# Autodesk Inventor assembly: p80 mount assembl
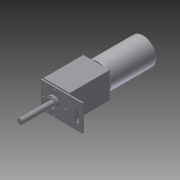
[picture p0: Inventor's stored thumbnail of the model, 180x180]
Saved by Autodesk Inventor 2013 (Build 170138000, 138)
## iProperties
Created: 2013-02-03
Part Number: p80 mount assembl
Document SubType Name: Assembly
Designer: Arpan
Mass: 804.871 g
Surface Area: 938.695 cm^2
Volume: 776.478 cm^3
Density: 1.03657 g/cm^3
Author: Arpan
## Documents named in this file (4)
- C:\Users\Moses\Documents\GitHub\frc2013CAD\Cimber actual\p80 mount assembl.iam
- C:\Users\Moses\Documents\GitHub\frc2013CAD\Cimber actual\p80 mount plate.ipt
- C:\Users\Moses\Documents\GitHub\frc2013CAD\Cimber actual\Cim and p80 rough.iam
- C:\Users\Moses\Documents\GitHub\frc2013CAD\Cimber actual\1.5 inch bearing.ipt
## Components (3 placed, 3 different names)
1. p80 mount plate:1 — Mate:1, Mate:2, Flush:1
2. Cim and p80 rough:1 [sub-assembly] — Mate:3, Flush:1, Mate:4
3. 1.5 inch bearing:1 — Mate:1, Mate:2, Mate:3, Mate:4
## Relationships (5: Mate 4, Flush 1)
- Mate:1: p80 mount plate:1 ↔ 1.5 inch bearing:1
- Mate:2: p80 mount plate:1 ↔ 1.5 inch bearing:1
- Mate:3: Cim and p80 rough:1 ↔ 1.5 inch bearing:1
- Flush:1: p80 mount plate:1 ↔ Cim and p80 rough:1
- Mate:4: Cim and p80 rough:1 ↔ 1.5 inch bearing:1
